# Autodesk Inventor assembly: Tie Rod Assembly
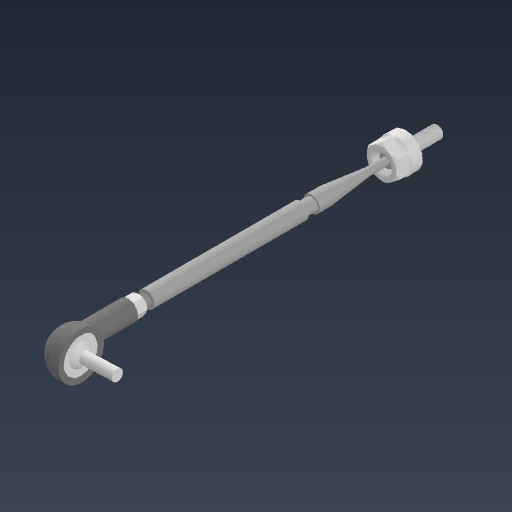
[picture p0: Inventor's stored thumbnail of the model, 512x512]
Saved by Autodesk Inventor 2021 (Build 250183000, 183)
## iProperties
Created: 2020-10-16
Part Number: Tie Rod Assembly
Document SubType Name: Assembly
Designer: Eugene Tang
Mass: 155.84 g
Surface Area: 593.185 cm^2
Volume: 155.84 cm^3
Density: 1 g/cm^3
Author: Eugene Tang
## Documents named in this file (8)
- C:\Users\teuge\OneDrive - Curtin University of Technology Australia\Y4S2\DFM\Group Project\CAD\Master\Tie Rod Assembly.iam
- C:\Users\teuge\OneDrive - Curtin University of Technology Australia\Y4S2\DFM\Group Project\CAD\Master\Inner Ball Joint (Body).ipt
- C:\Users\teuge\OneDrive - Curtin University of Technology Australia\Y4S2\DFM\Group Project\CAD\Master\Inner Ball Joint (Cap).ipt
- C:\Users\teuge\OneDrive - Curtin University of Technology Australia\Y4S2\DFM\Group Project\CAD\Master\Tie Rod.ipt
- C:\Users\teuge\OneDrive - Curtin University of Technology Australia\Y4S2\DFM\Group Project\CAD\Parts\Nut Fastener.ipt
- C:\Users\teuge\OneDrive - Curtin University of Technology Australia\Y4S2\DFM\Group Project\CAD\Parts\Out Tie Rod Joint Cap.ipt
- C:\Users\teuge\OneDrive - Curtin University of Technology Australia\Y4S2\DFM\Group Project\CAD\Parts\Outer Tie Rod Ball.ipt
- C:\Users\teuge\OneDrive - Curtin University of Technology Australia\Y4S2\DFM\Group Project\CAD\Parts\Outer Tie Rod.ipt
## Components (7 placed, 7 different names)
1. Inner Ball Joint (Body):1 — Mate:1, Mate:3
2. Inner Ball Joint (Cap):1 — Mate:1, Mate:2, Mate:3, Mate:4
3. Tie Rod:1 — Mate:2, Mate:4, Mate:5, Mate:6, Mate:7
4. Nut Fastener:1 — Mate:5, Mate:6, Mate:8
5. Out Tie Rod Joint Cap:1 — Mate:9, Mate:10
6. Outer Tie Rod Ball:1 — Mate:11
7. Outer Tie Rod:1 — Mate:7, Mate:8, Mate:9, Mate:10, Mate:11
## Relationships (11: Mate 11)
- Mate:1: Inner Ball Joint (Body):1 ↔ Inner Ball Joint (Cap):1
- Mate:2: Inner Ball Joint (Cap):1 ↔ Tie Rod:1
- Mate:3: Inner Ball Joint (Body):1 ↔ Inner Ball Joint (Cap):1
- Mate:4: Inner Ball Joint (Cap):1 ↔ Tie Rod:1
- Mate:5 (7.8 mm): Tie Rod:1 ↔ Nut Fastener:1
- Mate:6: Tie Rod:1 ↔ Nut Fastener:1
- Mate:7: Tie Rod:1 ↔ Outer Tie Rod:1
- Mate:8: Nut Fastener:1 ↔ Outer Tie Rod:1
- Mate:9: Out Tie Rod Joint Cap:1 ↔ Outer Tie Rod:1
- Mate:10: Out Tie Rod Joint Cap:1 ↔ Outer Tie Rod:1
- Mate:11: Outer Tie Rod Ball:1 ↔ Outer Tie Rod:1
